# Autodesk Inventor assembly: Montagem2
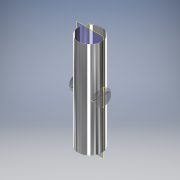
[picture p0: Inventor's stored thumbnail of the model, 180x180]
Saved by Autodesk Inventor 2016 (Build 200138000, 138)
## iProperties
Created: 2017-04-03
Part Number: Montagem2
Document SubType Name: Assembly
Designer: Marcelo
Author: Marcelo
## Documents named in this file (4)
- D:\Users\Marcelo\Documents\GitHub\telescopiocaseiro\Hardware\PT-001\Montagem2.iam
- D:\Users\Marcelo\Documents\GitHub\telescopiocaseiro\Hardware\PT-001\Tubo.ipt
- D:\Users\Marcelo\Documents\GitHub\telescopiocaseiro\Hardware\PT-001\DiscoSuporteInterno.ipt
- D:\Users\Marcelo\Documents\GitHub\telescopiocaseiro\Hardware\PT-001\DiscoSuporteExterno.ipt
## Components (5 placed, 3 different names)
1. Tubo:1 — Mate:1, Mate:4, Mate:10, Mate:11, Flush:1
2. DiscoSuporteInterno:1 — Mate:1, Mate:4, Mate:8, Mate:9
3. DiscoSuporteExterno:1 — Mate:8, Mate:9
4. DiscoSuporteExterno:2 — Mate:12, Mate:13
5. DiscoSuporteInterno:2 — Mate:10, Mate:11, Flush:1, Mate:12, Mate:13
## Relationships (9: Mate 8, Flush 1)
- Mate:1: Tubo:1 ↔ DiscoSuporteInterno:1
- Mate:4 (-400 mm): Tubo:1 ↔ DiscoSuporteInterno:1
- Mate:8: DiscoSuporteInterno:1 ↔ DiscoSuporteExterno:1
- Mate:9: DiscoSuporteInterno:1 ↔ DiscoSuporteExterno:1
- Mate:10: Tubo:1 ↔ DiscoSuporteInterno:2
- Mate:11 (-400 mm): Tubo:1 ↔ DiscoSuporteInterno:2
- Flush:1: Tubo:1 ↔ DiscoSuporteInterno:2
- Mate:12: DiscoSuporteExterno:2 ↔ DiscoSuporteInterno:2
- Mate:13: DiscoSuporteExterno:2 ↔ DiscoSuporteInterno:2
